# Autodesk Inventor assembly: Banebots RS-775 P60 Planetary Gearbox 64 to 1 (0.5x3 shaft)
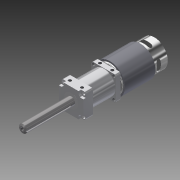
[picture p0: Inventor's stored thumbnail of the model, 180x180]
Saved by Autodesk Inventor 2013 (Build 170138000, 138)
## iProperties
Created: 2012-01-14
Part Number: Banebots RS-775 P60 Planetary Gearbox 64 to 1 (0.5x3 shaft)
Document SubType Name: Assembly
Designer: Moses
Mass: 816.466 g
Surface Area: 503.325 cm^2
Volume: 70.6506 cm^3
Author: Moses
## Documents named in this file (7)
- C:\Users\Moses\Documents\GitHub\frc2013CAD\M-Climber\Banebots P60\Banebots RS-775 P60 Planetary Gearbox 64 to 1 (0.5x3 shaft).iam
- C:\Users\Moses\Documents\GitHub\frc2013CAD\M-Climber\Banebots P60\Gearbox End Plate.ipt
- C:\Users\Moses\Documents\GitHub\frc2013CAD\M-Climber\Banebots P60\Gearbox End Plate 2.ipt
- C:\Users\Moses\Documents\GitHub\frc2013CAD\M-Climber\Banebots P60\R6Z Ball Bearing (0.375x0.875).ipt
- C:\Users\Moses\Documents\GitHub\frc2013CAD\M-Climber\Banebots P60\Banebots 0.5x3 P60 Shaft.ipt
- C:\Users\Moses\Documents\GitHub\frc2013CAD\M-Climber\Banebots P60\Motors_BaneBots_RS-775.ipt
- C:\Users\Moses\Documents\GitHub\frc2013CAD\M-Climber\Banebots P60\Gearbox Ring Gear 64 to 1.ipt
## Components (7 placed, 6 different names)
1. Gearbox End Plate:1 — Insert:2, Flush:1, Flush:2, Insert:4, Insert:5
2. Gearbox Ring Gear 64 to 1:1 — Insert:2, Insert:3
3. Gearbox End Plate 2:1 — Insert:3, Flush:1, Flush:2, Insert:7
4. R6Z Ball Bearing (0.375x0.875):1 — Insert:4
5. R6Z Ball Bearing (0.375x0.875):2 — Insert:5, Insert:6
6. Banebots 0.5x3 P60 Shaft:1 — Insert:6
7. Motors_BaneBots_RS-775:1 — Insert:7
## Relationships (8: Insert 6, Flush 2)
- Insert:2: Gearbox End Plate:1 ↔ Gearbox Ring Gear 64 to 1:1
- Insert:3: Gearbox Ring Gear 64 to 1:1 ↔ Gearbox End Plate 2:1
- Flush:1: Gearbox End Plate:1 ↔ Gearbox End Plate 2:1
- Flush:2: Gearbox End Plate:1 ↔ Gearbox End Plate 2:1
- Insert:4: Gearbox End Plate:1 ↔ R6Z Ball Bearing (0.375x0.875):1
- Insert:5: Gearbox End Plate:1 ↔ R6Z Ball Bearing (0.375x0.875):2
- Insert:6: R6Z Ball Bearing (0.375x0.875):2 ↔ Banebots 0.5x3 P60 Shaft:1
- Insert:7: Gearbox End Plate 2:1 ↔ Motors_BaneBots_RS-775:1
